# Autodesk Inventor assembly: cellSTORM_UC2_motorized_micrometer
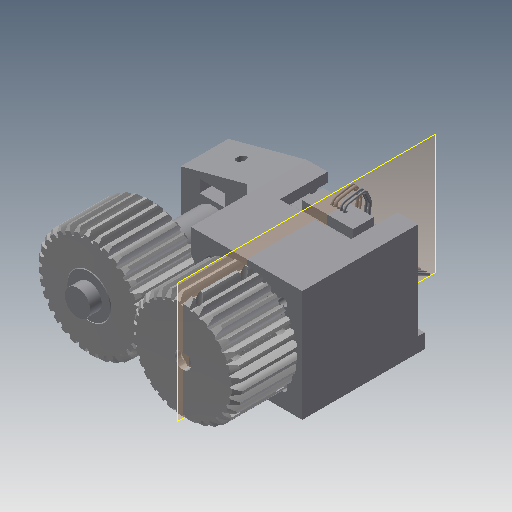
[picture p0: Inventor's stored thumbnail of the model, 512x512]
Saved by Autodesk Inventor 2019.4 (Build 234330000, 330)
## iProperties
Created: 2021-01-04
Part Number: cellSTORM_UC2_motorized_micrometer
Document SubType Name: Assembly
Designer: diederichbenedict
Author: diederichbenedict
## Documents named in this file (6)
- C:\Users\diederichbenedict\Dropbox\Dokumente\Promotion\PROJECTS\UC2\02_CAD\INVENTOR\uc2_v3\cellstrom\cellSTORM_UC2_motorized_micrometer.iam
- C:\Users\diederichbenedict\Dropbox\Dokumente\Promotion\PROJECTS\UC2\02_CAD\INVENTOR\uc2_v3\00_NEMA11.ipt
- C:\Users\diederichbenedict\Dropbox\Dokumente\Promotion\PROJECTS\UC2\02_CAD\INVENTOR\uc2_v3\00_micrometer_xy-stage.ipt
- C:\Users\diederichbenedict\Dropbox\Dokumente\Promotion\PROJECTS\UC2\02_CAD\INVENTOR\uc2_v3\cellstrom\cellSTORM_UC2_motorized_micrometer_gear1.ipt
- C:\Users\diederichbenedict\Dropbox\Dokumente\Promotion\PROJECTS\UC2\02_CAD\INVENTOR\uc2_v3\cellstrom\cellSTORM_UC2_motorized_micrometer_gear2.ipt
- C:\Users\diederichbenedict\Dropbox\Dokumente\Promotion\PROJECTS\UC2\02_CAD\INVENTOR\uc2_v3\cellstrom\cellSTORM_UC2_motorized_micrometer_motormount.ipt
## Components (5 placed, 4 different names)
1. 00_micrometer_xy-stage:1 — Mate:4, Mate:6
2. 00_NEMA11:1 — Mate:5, Mate:6, Mate:7, Flush:3
3. Spur Gear2:2 — Mate:5, Mate:7
4. Spur Gear2:3 — Mate:4
5. cellSTORM_UC2_motorized_micrometer_motormount:1 — Flush:3
## Relationships (8: Mate 5, Flush 3)
- [Mate] (32.2 mm): 00_micrometer_xy-stage:1 ↔ 00_NEMA11:1
- [Flush]: 00_micrometer_xy-stage:1 ↔ 00_NEMA11:1
- [Flush]: 00_micrometer_xy-stage:1 ↔ 00_NEMA11:1
- Mate:4: 00_micrometer_xy-stage:1 ↔ Spur Gear2:3
- Mate:5: 00_NEMA11:1 ↔ Spur Gear2:2
- Mate:6 (32.2 mm): 00_micrometer_xy-stage:1 ↔ 00_NEMA11:1
- Mate:7: 00_NEMA11:1 ↔ Spur Gear2:2
- Flush:3: 00_NEMA11:1 ↔ cellSTORM_UC2_motorized_micrometer_motormount:1
